# Autodesk Inventor assembly: Front Clear Door Assambly
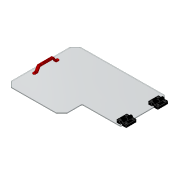
[picture p0: Inventor's stored thumbnail of the model, 180x180]
Saved by Autodesk Inventor 2015 (Build 190159000, 159)
## iProperties
Created: 2018-04-21
Part Number: Front Clear Door Assambly
Document SubType Name: Assembly
Designer: Ghassan Yusuf
Author: Ghassan Yusuf
## Documents named in this file (4)
- X:\TAKEONE\Products\takeone-3D-printer\model\3D\Front Clear Door Assambly.iam
- X:\TAKEONE\Products\takeone-3D-printer\model\3D\Clear Front Door.ipt
- X:\TAKEONE\Products\takeone-3D-printer\model\3D\Hing Assambly.iam
- X:\Autodesk Designs\MakerBot Transformation\Door Handle.ipt
## Components (4 placed, 3 different names)
1. Clear Front Door:1 — Insert:22, Insert:23, Insert:24, Insert:25, Insert:26, Insert:27
2. Hing Assambly:1 [sub-assembly] — Insert:22, Insert:23, Flush:1
3. Hing Assambly:2 [sub-assembly] — Insert:24, Insert:25, Flush:1
4. Door Handle:1 — Insert:26, Insert:27
## Relationships (7: Insert 6, Flush 1)
- Insert:22: Clear Front Door:1 ↔ Hing Assambly:1
- Insert:23: Clear Front Door:1 ↔ Hing Assambly:1
- Insert:24: Clear Front Door:1 ↔ Hing Assambly:2
- Insert:25: Clear Front Door:1 ↔ Hing Assambly:2
- Flush:1: Hing Assambly:1 ↔ Hing Assambly:2
- Insert:26: Clear Front Door:1 ↔ Door Handle:1
- Insert:27: Clear Front Door:1 ↔ Door Handle:1
